# Autodesk Inventor assembly: Assemblybearing
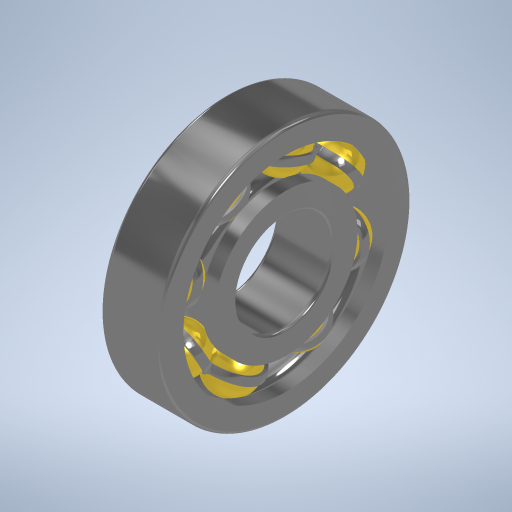
[picture p0: Inventor's stored thumbnail of the model, 512x512]
Saved by Autodesk Inventor 2023 (Build 270158000, 158)
## iProperties
Created: 2023-03-23
Part Number: Assemblybearing
Document SubType Name: Assembly
Designer: kaanf
Author: kaanf
## Documents named in this file (5)
- C:\Users\kaanf\Documents\Inventor\Assemblys\Assemblybearing.iam
- C:\Users\kaanf\Downloads\Outer Ring(fixed).ipt
- C:\Users\kaanf\Downloads\Inner Ring (2).ipt
- C:\Users\kaanf\Downloads\ball (2).ipt
- C:\Users\kaanf\Downloads\Cage (1).ipt
## Components (11 placed, 4 different names)
1. Outer Ring(fixed):1 — Mate:1, Flush:1, Mate:2
2. Inner Ring (2):1 — Mate:1, Flush:1, Tangent:1, Mate:3, Mate:5
3. Cage (1):1 — Mate:4, Mate:5, Mate:6
4. ball (2):1 — Mate:2, Tangent:1, Mate:3, Mate:6
5. ball (2):2
6. ball (2):3
7. ball (2):4
8. ball (2):5
9. ball (2):6
10. ball (2):7
11. ball (2):8
## Component patterns: (8 elements, first: ball (2):1)
## Relationships (8: Mate 6, Flush 1, Tangent 1)
- Mate:1: Outer Ring(fixed):1 ↔ Inner Ring (2):1
- Flush:1: Outer Ring(fixed):1 ↔ Inner Ring (2):1
- Mate:2: Outer Ring(fixed):1 ↔ ball (2):1
- Tangent:1: Inner Ring (2):1 ↔ ball (2):1
- Mate:3: Inner Ring (2):1 ↔ ball (2):1
- Mate:4: Cage (1):1
- Mate:5: Inner Ring (2):1 ↔ Cage (1):1
- Mate:6: Cage (1):1 ↔ ball (2):1
